# Autodesk Inventor assembly: front
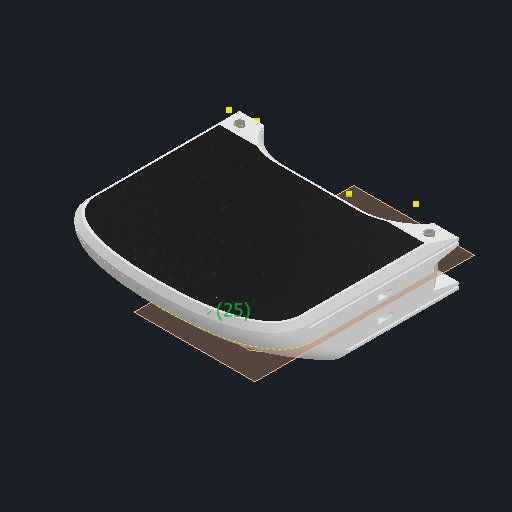
[picture p0: Inventor's stored thumbnail of the model, 512x512]
Saved by Autodesk Inventor 2025 (Build 290162000, 162)
## iProperties
Created: 2024-04-30
Part Number: front
Document SubType Name: Assembly
Designer: markm
Author: markm
## Documents named in this file (13)
- C:\Users\mark\OneDrive\Inventor\eventide\front\front.iam
- C:\Users\mark\OneDrive\Inventor\eventide\front\body.ipt
- C:\Users\mark\OneDrive\Inventor\eventide\front\esc.ipt
- C:\Users\mark\OneDrive\Inventor\eventide\front\cap.ipt
- C:\Users\mark\OneDrive\Inventor\Content Center Files\R2024\en-US\DIN 912\DIN 912 - M5 x 0,8 x 20 x 18.ipt
- C:\Users\mark\OneDrive\Inventor\eventide\front\pad.ipt
- C:\Users\mark\OneDrive\Inventor\eventide\front\pcb.ipt
- C:\Users\mark\OneDrive\Inventor\eventide\front\tenzo.ipt
- C:\Users\mark\OneDrive\Inventor\eventide\front\subcap.ipt
- C:\Users\mark\OneDrive\Inventor\eventide\front\Part1.ipt
- C:\Users\mark\OneDrive\Inventor\eventide\back\flank_MIR.ipt
- C:\Users\mark\OneDrive\Inventor\eventide\back\flank.ipt
- C:\Users\mark\OneDrive\Inventor\eventide\back\protection.ipt
## Components (23 placed, 12 different names)
1. body:1 — Flush:1, Flush:2, Mate:1, Mate:11, Mate:12, Mate:13, Mate:14, Mate:15, Mate:21, Mate:24, Flush:4, Mate:37, Mate:38, Flush:5, Mate:40, Mate:41, Mate:42
2. esc:1 — Mate:16, Mate:22
3. cap:1 — Flush:1, Flush:2, Mate:1, Mate:3, Mate:4, Mate:5, Mate:6, Mate:7, Mate:8, Mate:9, Mate:10, Mate:28, Mate:31, Mate:32, Mate:33, Mate:39
4. DIN 912 - replaced by DIN EN ISO 4762 M5 x 20:1 — Mate:5, Mate:6
5. DIN 912 - replaced by DIN EN ISO 4762 M5 x 20:2 — Mate:9, Mate:10
6. DIN 912 - replaced by DIN EN ISO 4762 M5 x 20:3 — Mate:13, Mate:14
7. DIN 912 - replaced by DIN EN ISO 4762 M5 x 20:4 — Mate:11, Mate:12
8. DIN 912 - replaced by DIN EN ISO 4762 M5 x 20:6 — Mate:7, Mate:8
9. DIN 912 - replaced by DIN EN ISO 4762 M5 x 20:7 — Mate:3, Mate:4
10. DIN 912 - replaced by DIN EN ISO 4762 M5 x 20:8
11. DIN 912 - replaced by DIN EN ISO 4762 M5 x 20:9
12. DIN 912 - replaced by DIN EN ISO 4762 M5 x 20:10
13. DIN 912 - replaced by DIN EN ISO 4762 M5 x 20:11
14. DIN 912 - replaced by DIN EN ISO 4762 M5 x 20:12
15. DIN 912 - replaced by DIN EN ISO 4762 M5 x 20:13
16. pad:1 — Mate:15, Mate:16, Mate:21, Mate:22, Mate:24
17. pcb:1
18. tenzo:1 — Mate:28, Mate:34, Mate:35, Mate:36
19. subcap:1 — Mate:31, Mate:32, Mate:33, Mate:34, Mate:35, Mate:36
20. Part1:1
21. flank_MIR:1 — Flush:4, Mate:37, Mate:38
22. flank:1 — Flush:5, Mate:39, Mate:40
23. protection:1 — Mate:41, Mate:42
## Relationships (35: Mate 31, Flush 4)
- Flush:1: body:1 ↔ cap:1
- Flush:2: body:1 ↔ cap:1
- Mate:1: body:1 ↔ cap:1
- Mate:3: cap:1 ↔ DIN 912 - replaced by DIN EN ISO 4762 M5 x 20:7
- Mate:4: cap:1 ↔ DIN 912 - replaced by DIN EN ISO 4762 M5 x 20:7
- Mate:5: cap:1 ↔ DIN 912 - replaced by DIN EN ISO 4762 M5 x 20:1
- Mate:6: cap:1 ↔ DIN 912 - replaced by DIN EN ISO 4762 M5 x 20:1
- Mate:7: cap:1 ↔ DIN 912 - replaced by DIN EN ISO 4762 M5 x 20:6
- Mate:8: cap:1 ↔ DIN 912 - replaced by DIN EN ISO 4762 M5 x 20:6
- Mate:9: cap:1 ↔ DIN 912 - replaced by DIN EN ISO 4762 M5 x 20:2
- Mate:10: cap:1 ↔ DIN 912 - replaced by DIN EN ISO 4762 M5 x 20:2
- Mate:11: body:1 ↔ DIN 912 - replaced by DIN EN ISO 4762 M5 x 20:4
- Mate:12: body:1 ↔ DIN 912 - replaced by DIN EN ISO 4762 M5 x 20:4
- Mate:13: body:1 ↔ DIN 912 - replaced by DIN EN ISO 4762 M5 x 20:3
- Mate:14: body:1 ↔ DIN 912 - replaced by DIN EN ISO 4762 M5 x 20:3
- Mate:15: body:1 ↔ pad:1
- Mate:16: esc:1 ↔ pad:1
- Mate:21: body:1 ↔ pad:1
- Mate:22: esc:1 ↔ pad:1
- Mate:24: body:1 ↔ pad:1
- Mate:28: cap:1 ↔ tenzo:1
- Mate:31: cap:1 ↔ subcap:1
- Mate:32: cap:1 ↔ subcap:1
- Mate:33: cap:1 ↔ subcap:1
- Mate:34: tenzo:1 ↔ subcap:1
- Mate:35: tenzo:1 ↔ subcap:1
- Mate:36: tenzo:1 ↔ subcap:1
- Flush:4: body:1 ↔ flank_MIR:1
- Mate:37 (1.5 mm): body:1 ↔ flank_MIR:1
- Mate:38 (1.5 mm): body:1 ↔ flank_MIR:1
- Flush:5: body:1 ↔ flank:1
- Mate:39 (1.5 mm): cap:1 ↔ flank:1
- Mate:40 (1.5 mm): body:1 ↔ flank:1
- Mate:41: body:1 ↔ protection:1
- Mate:42: body:1 ↔ protection:1
